# Autodesk Inventor assembly: buggy-assembly-group2
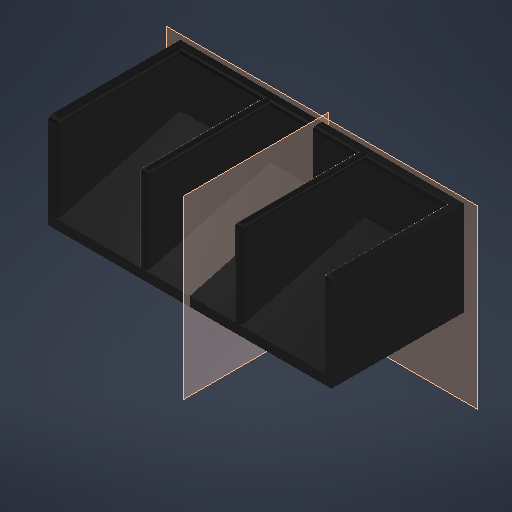
[picture p0: Inventor's stored thumbnail of the model, 512x512]
Saved by Autodesk Inventor 2026.1 (Build 301233000, 233)
## iProperties
Created: 2026-02-23
Part Number: buggy-assembly-group2
Document SubType Name: Assembly
Designer: ts2104
Author: ts2104
## Documents named in this file (2)
- C:\Users\ts2104\Documents\GitHub\System-Project-G2\mechanical\buggy-assembly-group2.iam
- C:\Users\ts2104\Documents\GitHub\System-Project-G2\mechanical\rubbish-container-group2.ipt
## Components (1 placed, 1 different names)
1. rubbish-container-group2:1 — Mate:1, Mate:2
## Relationships (2: Mate 2)
- Mate:1: rubbish-container-group2:1
- Mate:2: rubbish-container-group2:1
